# Autodesk Inventor assembly: CLB_030_ScissorLiftSliderFourPart
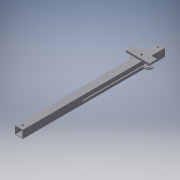
[picture p0: Inventor's stored thumbnail of the model, 180x180]
Saved by Autodesk Inventor 2018.3 (Build 223284000, 284)
## iProperties
Created: 2020-01-24
Part Number: CLB_030_ScissorLiftSliderFourPart
Document SubType Name: Assembly
Designer: Cooper
Author: Cooper
## Documents named in this file (4)
- C:\Users\22perngrac\Documents\GrabCAD\Infinite Recharge 2020\Build season\CLB_054_ScissorSliderFourPart.iam
- C:\Users\22perngrac\Documents\GrabCAD\Infinite Recharge 2020\Build season\CLB_032_ScissorLiftSliderWheel.ipt
- C:\Users\22perngrac\Documents\GrabCAD\Infinite Recharge 2020\Build season\CLB_033_ScissorLiftSliderBracket.ipt
- C:\Users\22perngrac\Documents\GrabCAD\Infinite Recharge 2020\Build season\CLB_031_ScissorLiftBase19.ipt
## Components (4 placed, 3 different names)
1. CLB_031_ScissorLiftBase19:1 — Mate:1, Mate:2, Flush:1, Angle:1, Tangent:1, Mate:3, Flush:2
2. CLB_032_ScissorLiftSliderWheel:1 — Insert:1, Tangent:1, Mate:3
3. CLB_032_ScissorLiftSliderWheel:2 — Insert:2
4. CLB_033_ScissorLiftSliderBracket:1 — Insert:1, Insert:2, Angle:1, Flush:2
## Relationships (9: Mate 3, Insert 2, Flush 2, Angle 1, Tangent 1)
- Insert:1: CLB_032_ScissorLiftSliderWheel:1 ↔ CLB_033_ScissorLiftSliderBracket:1
- Insert:2: CLB_032_ScissorLiftSliderWheel:2 ↔ CLB_033_ScissorLiftSliderBracket:1
- Mate:1: CLB_031_ScissorLiftBase19:1
- Mate:2: CLB_031_ScissorLiftBase19:1
- Flush:1: CLB_031_ScissorLiftBase19:1
- Angle:1 (0 deg): CLB_031_ScissorLiftBase19:1 ↔ CLB_033_ScissorLiftSliderBracket:1
- Tangent:1: CLB_031_ScissorLiftBase19:1 ↔ CLB_032_ScissorLiftSliderWheel:1
- Mate:3: CLB_031_ScissorLiftBase19:1 ↔ CLB_032_ScissorLiftSliderWheel:1
- Flush:2 (25.4 mm): CLB_031_ScissorLiftBase19:1 ↔ CLB_033_ScissorLiftSliderBracket:1
